# Autodesk Inventor assembly: airhockeybot_table_simulation
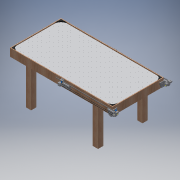
[picture p0: Inventor's stored thumbnail of the model, 180x180]
Saved by Autodesk Inventor 2019.3 (Build 233278000, 278)
## iProperties
Created: 2020-08-23
Part Number: airhockeybot_table_simulation
Material: Generisch
Document SubType Name: Assembly
Designer: Nicolas Frick
Author: Nicolas Frick
## Documents named in this file (22)
- C:\Users\Nicolas Frick\Sync\OneDrive\airhockeybot\mechanical_design\inventor\airhockeybot_table_simulation.iam
- C:\Users\Nicolas Frick\Sync\OneDrive\airhockeybot\mechanical_design\inventor\Table\Table.iam
- C:\Users\Nicolas Frick\Sync\OneDrive\airhockeybot\mechanical_design\inventor\Pulley.iam
- C:\Users\Nicolas Frick\Sync\OneDrive\airhockeybot\mechanical_design\inventor\Fixture_mid.ipt
- C:\Users\Nicolas Frick\Sync\OneDrive\airhockeybot\mechanical_design\inventor\Fixture_linear_mid.ipt
- C:\Users\Nicolas Frick\Sync\OneDrive\airhockeybot\mechanical_design\inventor\Bearing_support_outside.ipt
- C:\Users\Nicolas Frick\Sync\OneDrive\airhockeybot\mechanical_design\inventor\Bearing_support_inside.ipt
- C:\Users\Nicolas Frick\Sync\OneDrive\airhockeybot\mechanical_design\inventor\igus\EEWM_12_200_2.ipt
- C:\Users\Nicolas Frick\Sync\OneDrive\airhockeybot\mechanical_design\inventor\Switch CMV101D\CNDT_CMV101D.ipt
- C:\Users\Nicolas Frick\Sync\OneDrive\airhockeybot\mechanical_design\inventor\PowerS.ipt
- C:\Users\Nicolas Frick\Sync\OneDrive\airhockeybot\mechanical_design\inventor\PowerS_case.ipt
- C:\Users\Nicolas Frick\Sync\OneDrive\airhockeybot\mechanical_design\inventor\Cable_clamp.ipt
- C:\Users\Nicolas Frick\Sync\OneDrive\airhockeybot\mechanical_design\inventor\PowerS_cap.ipt
- C:\Users\Nicolas Frick\Sync\OneDrive\airhockeybot\mechanical_design\inventor\Nema 17HS5425\Assembly1.iam
- C:\Users\Nicolas Frick\Sync\OneDrive\airhockeybot\mechanical_design\inventor\GT2 40T 5mm Bore 6mm wide pulley\GT2 40T 5 Bore v2.iam
- C:\Users\Nicolas Frick\Sync\OneDrive\airhockeybot\mechanical_design\inventor\Fixture_linear_end.ipt
- C:\Users\Nicolas Frick\Sync\OneDrive\airhockeybot\mechanical_design\inventor\Fixture_motor.ipt
- C:\Users\Nicolas Frick\Sync\OneDrive\airhockeybot\mechanical_design\inventor\GT2 Belt 6mm\GT2 Belt 6mm x 40mm.ipt
- C:\Users\Nicolas Frick\Sync\OneDrive\airhockeybot\mechanical_design\inventor\Fixture_mid_right.ipt
- C:\Users\Nicolas Frick\Sync\OneDrive\airhockeybot\mechanical_design\inventor\Fixture_linear_mid_right.ipt
- C:\Users\Nicolas Frick\Sync\OneDrive\airhockeybot\mechanical_design\inventor\Fixture_motor_right.ipt
- C:\Users\Nicolas Frick\Sync\OneDrive\airhockeybot\mechanical_design\inventor\Fixture_linear_end_right.ipt
## Components (123 placed, 21 different names)
1. Table:1 [sub-assembly] — Fluchtend:1, Passend:1, Passend:2, Passend:5, Fluchtend:2, Fluchtend:3, Fluchtend:4, Passend:35, Passend:36, Passend:37, Passend:42, Passend:43, Fluchtend:26, Passend:69, Passend:70, Passend:86, Passend:87
2. Fixture_mid:1 — Fluchtend:1, Passend:1, Passend:2, Passend:3, Passend:4, Passend:6, Passend:7, Fluchtend:27, Fluchtend:28
3. Fixture_linear_mid:1 — Passend:3, Passend:4, Passend:5, Passend:23, Fluchtend:6
4. Bearing_support_outside:1 — Passend:10, Passend:11, Passend:12, Fluchtend:15, Passend:62, Passend:65, Fluchtend:25, Passend:66
5. Bearing_support_inside:1 — Passend:6, Passend:7, Passend:10, Passend:11, Passend:12, Fluchtend:24, Passend:63, Passend:67
6. EEWM_12_200_2:1 — Passend:41, Fluchtend:72
7. CNDT_CMV101D:1 — Passend:23, Fluchtend:6
8. PowerS:1 — Fluchtend:8, Fluchtend:11, Fluchtend:12, Passend:36, Passend:37
9. PowerS_case:1 — Fluchtend:8, Passend:31, Fluchtend:9, Fluchtend:10, Passend:32, Passend:33, Passend:34, Fluchtend:11, Fluchtend:12, Passend:35
10. Cable_clamp:1 — Passend:31, Fluchtend:9, Fluchtend:10
11. PowerS_cap:1 — Passend:32, Passend:33, Passend:34
12. Assembly1:1 [sub-assembly] — Passend:38, Fluchtend:15, Passend:44, Passend:58, Passend:68
13. GT2 40T 5 Bore v2:1 [sub-assembly] — Passend:38, Passend:68
14. Fixture_linear_end:1 — Passend:39, Fluchtend:17, Passend:41, Passend:46, Fluchtend:19, Fluchtend:22, Passend:59, Fluchtend:72
15. Fixture_motor:1 — Passend:39, Fluchtend:17, Passend:42, Passend:43, Passend:44, Passend:58, Passend:59, Fluchtend:29
16. CNDT_CMV101D:2 — Passend:46, Fluchtend:19, Fluchtend:22
17. Pulley:1 [sub-assembly] — Passend:66, Passend:67
18. Fixture_mid_right:1 — Passend:69, Fluchtend:27, Fluchtend:28, Passend:71, Passend:72, Passend:73, Passend:75
19. Fixture_linear_mid_right:1 — Passend:70, Passend:71, Passend:72, Passend:186
20. Bearing_support_inside:2 — Passend:73, Passend:75, Passend:77, Passend:78, Passend:79, Passend:81, Passend:101, Passend:103, Fluchtend:34
21. Bearing_support_outside:2 — Passend:78, Passend:80, Passend:81, Passend:100, Fluchtend:33, Passend:102
22. Pulley:2 [sub-assembly] — Passend:77, Passend:79, Passend:80
23. EEWM_12_200_2:2 — Passend:88, Passend:186, Fluchtend:71
24. Fixture_motor_right:1 — Passend:86, Fluchtend:29, Passend:87, Passend:89, Passend:90, Passend:95, Passend:96, Passend:104
25. Fixture_linear_end_right:1 — Passend:88, Passend:89, Passend:90, Fluchtend:71
26. Assembly1:2 [sub-assembly] — Passend:95, Passend:96, Passend:97, Fluchtend:32, Passend:104
27. GT2 40T 5 Bore v2:2 [sub-assembly] — Passend:97, Fluchtend:32
28. GT2 Belt 6mm x 40mm:1 — Fluchtend:24, Passend:63
29. GT2 Belt 6mm x 40mm:2 — Passend:62
30. GT2 Belt 6mm x 40mm:3
31. GT2 Belt 6mm x 40mm:4
32. GT2 Belt 6mm x 40mm:5
33. GT2 Belt 6mm x 40mm:6
34. GT2 Belt 6mm x 40mm:7
35. GT2 Belt 6mm x 40mm:8
36. GT2 Belt 6mm x 40mm:9
37. GT2 Belt 6mm x 40mm:10
38. GT2 Belt 6mm x 40mm:11
39. GT2 Belt 6mm x 40mm:12
40. GT2 Belt 6mm x 40mm:13
41. GT2 Belt 6mm x 40mm:14
42. GT2 Belt 6mm x 40mm:15
43. GT2 Belt 6mm x 40mm:16
44. GT2 Belt 6mm x 40mm:17
45. GT2 Belt 6mm x 40mm:18
46. GT2 Belt 6mm x 40mm:19
47. GT2 Belt 6mm x 40mm:20
48. GT2 Belt 6mm x 40mm:21
49. GT2 Belt 6mm x 40mm:22
50. GT2 Belt 6mm x 40mm:23
51. GT2 Belt 6mm x 40mm:24
52. GT2 Belt 6mm x 40mm:25 — Passend:65, Fluchtend:25
53. GT2 Belt 6mm x 40mm:26
54. GT2 Belt 6mm x 40mm:27
55. GT2 Belt 6mm x 40mm:28
56. GT2 Belt 6mm x 40mm:29
57. GT2 Belt 6mm x 40mm:30
58. GT2 Belt 6mm x 40mm:31
59. GT2 Belt 6mm x 40mm:32 — Fluchtend:26
60. GT2 Belt 6mm x 40mm:33
61. GT2 Belt 6mm x 40mm:34
62. GT2 Belt 6mm x 40mm:35
63. GT2 Belt 6mm x 40mm:36
64. GT2 Belt 6mm x 40mm:37
65. GT2 Belt 6mm x 40mm:38
66. GT2 Belt 6mm x 40mm:39
67. GT2 Belt 6mm x 40mm:40
68. GT2 Belt 6mm x 40mm:41
69. GT2 Belt 6mm x 40mm:42
70. GT2 Belt 6mm x 40mm:43
71. GT2 Belt 6mm x 40mm:44
72. GT2 Belt 6mm x 40mm:45
73. GT2 Belt 6mm x 40mm:46
74. GT2 Belt 6mm x 40mm:47
75. GT2 Belt 6mm x 40mm:48
76. GT2 Belt 6mm x 40mm:49 — Passend:100, Passend:101, Fluchtend:33
77. GT2 Belt 6mm x 40mm:51
78. GT2 Belt 6mm x 40mm:52
79. GT2 Belt 6mm x 40mm:53
80. GT2 Belt 6mm x 40mm:54
81. GT2 Belt 6mm x 40mm:55
82. GT2 Belt 6mm x 40mm:56
83. GT2 Belt 6mm x 40mm:57
84. GT2 Belt 6mm x 40mm:58
85. GT2 Belt 6mm x 40mm:59
86. GT2 Belt 6mm x 40mm:60
87. GT2 Belt 6mm x 40mm:61
88. GT2 Belt 6mm x 40mm:62
89. GT2 Belt 6mm x 40mm:63
90. GT2 Belt 6mm x 40mm:64
91. GT2 Belt 6mm x 40mm:65
92. GT2 Belt 6mm x 40mm:66
93. GT2 Belt 6mm x 40mm:67
94. GT2 Belt 6mm x 40mm:68
95. GT2 Belt 6mm x 40mm:69
96. GT2 Belt 6mm x 40mm:70
97. GT2 Belt 6mm x 40mm:71
98. GT2 Belt 6mm x 40mm:72
99. GT2 Belt 6mm x 40mm:73
100. GT2 Belt 6mm x 40mm:50 — Passend:102, Passend:103, Fluchtend:34
101. GT2 Belt 6mm x 40mm:74
102. GT2 Belt 6mm x 40mm:75
103. GT2 Belt 6mm x 40mm:76
104. GT2 Belt 6mm x 40mm:77
105. GT2 Belt 6mm x 40mm:78
106. GT2 Belt 6mm x 40mm:79
107. GT2 Belt 6mm x 40mm:80
108. GT2 Belt 6mm x 40mm:81
109. GT2 Belt 6mm x 40mm:82
110. GT2 Belt 6mm x 40mm:83
111. GT2 Belt 6mm x 40mm:84
112. GT2 Belt 6mm x 40mm:85
113. GT2 Belt 6mm x 40mm:86
114. GT2 Belt 6mm x 40mm:87
115. GT2 Belt 6mm x 40mm:88
116. GT2 Belt 6mm x 40mm:89
117. GT2 Belt 6mm x 40mm:90
118. GT2 Belt 6mm x 40mm:91
119. GT2 Belt 6mm x 40mm:92
120. GT2 Belt 6mm x 40mm:93
121. GT2 Belt 6mm x 40mm:94
122. GT2 Belt 6mm x 40mm:95
123. GT2 Belt 6mm x 40mm:96
## Component patterns: (24 elements, first: GT2 Belt 6mm x 40mm:1), (24 elements, first: GT2 Belt 6mm x 40mm:25), (24 elements, first: GT2 Belt 6mm x 40mm:49), (24 elements, first: GT2 Belt 6mm x 40mm:50)
## Relationships (83: Mate 58, Flush 25)
- Fluchtend:1 [Flush] (747.832 mm): Table:1 ↔ Fixture_mid:1
- Passend:1 [Mate]: Table:1 ↔ Fixture_mid:1
- Passend:2 [Mate] (74 mm): Table:1 ↔ Fixture_mid:1
- Passend:3 [Mate]: Fixture_mid:1 ↔ Fixture_linear_mid:1
- Passend:4 [Mate]: Fixture_mid:1 ↔ Fixture_linear_mid:1
- Passend:5 [Mate]: Table:1 ↔ Fixture_linear_mid:1
- Fluchtend:2 [Flush]: Table:1
- Fluchtend:3 [Flush]: Table:1
- Fluchtend:4 [Flush]: Table:1
- Passend:6 [Mate] (0.05 mm): Fixture_mid:1 ↔ Bearing_support_inside:1
- Passend:7 [Mate] (0.05 mm): Fixture_mid:1 ↔ Bearing_support_inside:1
- Passend:10 [Mate]: Bearing_support_outside:1 ↔ Bearing_support_inside:1
- Passend:11 [Mate]: Bearing_support_outside:1 ↔ Bearing_support_inside:1
- Passend:12 [Mate]: Bearing_support_outside:1 ↔ Bearing_support_inside:1
- Passend:23 [Mate]: Fixture_linear_mid:1 ↔ CNDT_CMV101D:1
- Fluchtend:6 [Flush]: Fixture_linear_mid:1 ↔ CNDT_CMV101D:1
- Fluchtend:8 [Flush]: PowerS:1 ↔ PowerS_case:1
- Passend:31 [Mate]: PowerS_case:1 ↔ Cable_clamp:1
- Fluchtend:9 [Flush]: PowerS_case:1 ↔ Cable_clamp:1
- Fluchtend:10 [Flush]: PowerS_case:1 ↔ Cable_clamp:1
- Passend:32 [Mate]: PowerS_case:1 ↔ PowerS_cap:1
- Passend:33 [Mate]: PowerS_case:1 ↔ PowerS_cap:1
- Passend:34 [Mate]: PowerS_case:1 ↔ PowerS_cap:1
- Fluchtend:11 [Flush]: PowerS:1 ↔ PowerS_case:1
- Fluchtend:12 [Flush]: PowerS:1 ↔ PowerS_case:1
- Passend:35 [Mate]: Table:1 ↔ PowerS_case:1
- Passend:36 [Mate] (50 mm): Table:1 ↔ PowerS:1
- Passend:37 [Mate] (250 mm): Table:1 ↔ PowerS:1
- Passend:38 [Mate]: Assembly1:1 ↔ GT2 40T 5 Bore v2:1
- Fluchtend:15 [Flush] (3.85 mm): Bearing_support_outside:1 ↔ Assembly1:1
- Passend:39 [Mate]: Fixture_linear_end:1 ↔ Fixture_motor:1
- Fluchtend:17 [Flush]: Fixture_linear_end:1 ↔ Fixture_motor:1
- Passend:41 [Mate]: EEWM_12_200_2:1 ↔ Fixture_linear_end:1
- Passend:42 [Mate]: Table:1 ↔ Fixture_motor:1
- Passend:43 [Mate]: Table:1 ↔ Fixture_motor:1
- Passend:44 [Mate]: Assembly1:1 ↔ Fixture_motor:1
- Passend:46 [Mate]: Fixture_linear_end:1 ↔ CNDT_CMV101D:2
- Fluchtend:19 [Flush] (12 mm): Fixture_linear_end:1 ↔ CNDT_CMV101D:2
- Passend:58 [Mate] (0.15 mm): Assembly1:1 ↔ Fixture_motor:1
- Fluchtend:22 [Flush] (4 mm): Fixture_linear_end:1 ↔ CNDT_CMV101D:2
- Passend:59 [Mate]: Fixture_linear_end:1 ↔ Fixture_motor:1
- Passend:62 [Mate] (2.7 mm): Bearing_support_outside:1 ↔ GT2 Belt 6mm x 40mm:2
- Fluchtend:24 [Flush] (16.1 mm): Bearing_support_inside:1 ↔ GT2 Belt 6mm x 40mm:1
- Passend:63 [Mate] (12.7 mm): Bearing_support_inside:1 ↔ GT2 Belt 6mm x 40mm:1
- Passend:65 [Mate] (5.5 mm): Bearing_support_outside:1 ↔ GT2 Belt 6mm x 40mm:25
- Fluchtend:25 [Flush] (15 mm): Bearing_support_outside:1 ↔ GT2 Belt 6mm x 40mm:25
- Fluchtend:26 [Flush] (52 mm): Table:1 ↔ GT2 Belt 6mm x 40mm:32
- Passend:66 [Mate]: Bearing_support_outside:1 ↔ Pulley:1
- Passend:67 [Mate]: Bearing_support_inside:1 ↔ Pulley:1
- Passend:68 [Mate] (2.5 mm): Assembly1:1 ↔ GT2 40T 5 Bore v2:1
- Passend:69 [Mate]: Table:1 ↔ Fixture_mid_right:1
- Fluchtend:27 [Flush]: Fixture_mid:1 ↔ Fixture_mid_right:1
- Fluchtend:28 [Flush]: Fixture_mid:1 ↔ Fixture_mid_right:1
- Passend:70 [Mate]: Table:1 ↔ Fixture_linear_mid_right:1
- Passend:71 [Mate]: Fixture_mid_right:1 ↔ Fixture_linear_mid_right:1
- Passend:72 [Mate]: Fixture_mid_right:1 ↔ Fixture_linear_mid_right:1
- Passend:73 [Mate]: Fixture_mid_right:1 ↔ Bearing_support_inside:2
- Passend:75 [Mate] (0.1 mm): Fixture_mid_right:1 ↔ Bearing_support_inside:2
- Passend:77 [Mate]: Bearing_support_inside:2 ↔ Pulley:2
- Passend:78 [Mate]: Bearing_support_inside:2 ↔ Bearing_support_outside:2
- Passend:79 [Mate]: Bearing_support_inside:2 ↔ Pulley:2
- Passend:80 [Mate]: Bearing_support_outside:2 ↔ Pulley:2
- Passend:81 [Mate]: Bearing_support_inside:2 ↔ Bearing_support_outside:2
- Passend:86 [Mate]: Table:1 ↔ Fixture_motor_right:1
- Fluchtend:29 [Flush]: Fixture_motor:1 ↔ Fixture_motor_right:1
- Passend:87 [Mate]: Table:1 ↔ Fixture_motor_right:1
- Passend:88 [Mate]: EEWM_12_200_2:2 ↔ Fixture_linear_end_right:1
- Passend:89 [Mate]: Fixture_motor_right:1 ↔ Fixture_linear_end_right:1
- Passend:90 [Mate]: Fixture_motor_right:1 ↔ Fixture_linear_end_right:1
- Passend:95 [Mate]: Fixture_motor_right:1 ↔ Assembly1:2
- Passend:96 [Mate]: Fixture_motor_right:1 ↔ Assembly1:2
- Passend:97 [Mate]: Assembly1:2 ↔ GT2 40T 5 Bore v2:2
- Fluchtend:32 [Flush] (-3 mm): Assembly1:2 ↔ GT2 40T 5 Bore v2:2
- Passend:100 [Mate] (2.5 mm): Bearing_support_outside:2 ↔ GT2 Belt 6mm x 40mm:49
- Passend:101 [Mate] (12.8 mm): Bearing_support_inside:2 ↔ GT2 Belt 6mm x 40mm:49
- Fluchtend:33 [Flush] (20 mm): Bearing_support_outside:2 ↔ GT2 Belt 6mm x 40mm:49
- Passend:102 [Mate] (2.5 mm): Bearing_support_outside:2 ↔ GT2 Belt 6mm x 40mm:50
- Passend:103 [Mate] (12.8 mm): Bearing_support_inside:2 ↔ GT2 Belt 6mm x 40mm:50
- Fluchtend:34 [Flush] (20 mm): Bearing_support_inside:2 ↔ GT2 Belt 6mm x 40mm:50
- Passend:104 [Mate] (3.984 mm): Fixture_motor_right:1 ↔ Assembly1:2
- Passend:186 [Mate]: Fixture_linear_mid_right:1 ↔ EEWM_12_200_2:2
- Fluchtend:71 [Flush]: EEWM_12_200_2:2 ↔ Fixture_linear_end_right:1
- Fluchtend:72 [Flush]: EEWM_12_200_2:1 ↔ Fixture_linear_end:1
